# Autodesk Inventor assembly: Y Axis Assembly 1.0_MIR
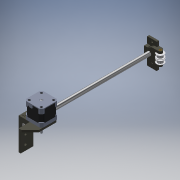
[picture p0: Inventor's stored thumbnail of the model, 180x180]
Saved by Autodesk Inventor 2016 (Build 200138000, 138)
## iProperties
Created: 2017-04-09
Part Number: Y Axis Assembly 1.0_MIR
Document SubType Name: Assembly
Designer: Scott
Author: Scott
## Documents named in this file (11)
- E:\Scott Projects\3D Printing\CoreXY\Y Axis Assembly 1.0_MIR.iam
- E:\Scott Projects\3D Printing\CoreXY\Linear rail - Y_MIR.ipt
- E:\Scott Projects\3D Printing\CoreXY\XY Idler Mount 1.0_MIR.ipt
- E:\Scott Projects\3D Printing\CoreXY\XY Stepper Mount 1.0_MIR.ipt
- E:\Scott Projects\3D Printing\CoreXY\M3 Threaded Insert_MIR3.ipt
- C:\Users\Scott\Documents\Inventor\Content Center Files\R2016\en-US\ANSI B18.3.1M(1)\ANSI B18.3.1M - M3x0.5 x 20(2).ipt
- C:\Users\Scott\Documents\Inventor\Content Center Files\R2016\en-US\ANSI B18.3.1M(1)\ANSI B18.3.1M - M3x0.5 x 30(2).ipt
- E:\Scott Projects\3D Printing\CoreXY\GT2_20t_wheel_pulley_MIR2.ipt
- C:\Users\Scott\Documents\Inventor\Content Center Files\R2016\en-US\ISO 7089\ISO 7089 - 3 - 140 HV(1).ipt
- C:\Users\Scott\Documents\Inventor\Content Center Files\R2016\en-US\AS 1420\AS 1420 - 1973 - M3 x 12.ipt
- E:\Scott Projects\3D Printing\CoreXY\NEMA 17 Stepper Motor Assembly.iam
## Components (19 placed, 10 different names)
1. Linear rail - Y_MIR:1 — Flush:3, Flush:2, Flush:1, Angle:1, Mate:1, Flush:4, Mate:2, Flush:5
2. XY Idler Mount 1.0_MIR:1 — Angle:1, Mate:1, Flush:4, Angle:2, Insert:2, Insert:3, Insert:5, Insert:6, Insert:7, Insert:8
3. XY Stepper Mount 1.0_MIR:1 — Angle:2, Mate:2, Flush:5, Insert:1, Insert:4, Insert:16, Insert:15, Insert:14, Insert:17, Angle:3
4. M3 Threaded Insert_MIR3:1 — Insert:2
5. M3 Threaded Insert_MIR3:2 — Insert:3
6. M3 Threaded Insert_MIR3:3 — Insert:1
7. Broached Socket Head Cap Screw - Metric M3x0.5 x 20:1 — Insert:4
8. Broached Socket Head Cap Screw - Metric M3x0.5 x 20:2 — Insert:5
9. Broached Socket Head Cap Screw - Metric M3x0.5 x 30:1 — Insert:6
10. GT2_20t_wheel_pulley_MIR2:1 — Insert:7, Insert:9
11. GT2_20t_wheel_pulley_MIR2:2 — Insert:8
12. ISO 7089 3 - 140 HV:1 — Insert:9, Insert:10
13. ISO 7089 3 - 140 HV:2 — Insert:12
14. ISO 7089 3 - 140 HV:3 — Insert:12, Insert:11
15. ISO 7089 3 - 140 HV:4 — Insert:11, Insert:10
16. AS 1420 - Metric M3 x 12:1 — Insert:16
17. AS 1420 - Metric M3 x 12:2 — Insert:15
18. AS 1420 - Metric M3 x 12:3 — Insert:14
19. NEMA 17 Stepper Motor Assembly:1 [sub-assembly] — Insert:17, Angle:3
## Relationships (26: Insert 16, Flush 5, Angle 3, Mate 2)
- Flush:3: Linear rail - Y_MIR:1
- Flush:2: Linear rail - Y_MIR:1
- Flush:1: Linear rail - Y_MIR:1
- Angle:1 (180 deg): Linear rail - Y_MIR:1 ↔ XY Idler Mount 1.0_MIR:1
- Mate:1: Linear rail - Y_MIR:1 ↔ XY Idler Mount 1.0_MIR:1
- Flush:4: Linear rail - Y_MIR:1 ↔ XY Idler Mount 1.0_MIR:1
- Angle:2 (0 deg): XY Idler Mount 1.0_MIR:1 ↔ XY Stepper Mount 1.0_MIR:1
- Mate:2: Linear rail - Y_MIR:1 ↔ XY Stepper Mount 1.0_MIR:1
- Flush:5: Linear rail - Y_MIR:1 ↔ XY Stepper Mount 1.0_MIR:1
- Insert:2: XY Idler Mount 1.0_MIR:1 ↔ M3 Threaded Insert_MIR3:1
- Insert:3: XY Idler Mount 1.0_MIR:1 ↔ M3 Threaded Insert_MIR3:2
- Insert:1: XY Stepper Mount 1.0_MIR:1 ↔ M3 Threaded Insert_MIR3:3
- Insert:4: XY Stepper Mount 1.0_MIR:1 ↔ Broached Socket Head Cap Screw - Metric M3x0.5 x 20:1
- Insert:5: XY Idler Mount 1.0_MIR:1 ↔ Broached Socket Head Cap Screw - Metric M3x0.5 x 20:2
- Insert:6: XY Idler Mount 1.0_MIR:1 ↔ Broached Socket Head Cap Screw - Metric M3x0.5 x 30:1
- Insert:7: XY Idler Mount 1.0_MIR:1 ↔ GT2_20t_wheel_pulley_MIR2:1
- Insert:8: XY Idler Mount 1.0_MIR:1 ↔ GT2_20t_wheel_pulley_MIR2:2
- Insert:9: GT2_20t_wheel_pulley_MIR2:1 ↔ ISO 7089 3 - 140 HV:1
- Insert:12: ISO 7089 3 - 140 HV:2 ↔ ISO 7089 3 - 140 HV:3
- Insert:11: ISO 7089 3 - 140 HV:3 ↔ ISO 7089 3 - 140 HV:4
- Insert:10: ISO 7089 3 - 140 HV:1 ↔ ISO 7089 3 - 140 HV:4
- Insert:16: XY Stepper Mount 1.0_MIR:1 ↔ AS 1420 - Metric M3 x 12:1
- Insert:15: XY Stepper Mount 1.0_MIR:1 ↔ AS 1420 - Metric M3 x 12:2
- Insert:14: XY Stepper Mount 1.0_MIR:1 ↔ AS 1420 - Metric M3 x 12:3
- Insert:17: XY Stepper Mount 1.0_MIR:1 ↔ NEMA 17 Stepper Motor Assembly:1
- Angle:3 (0 deg): XY Stepper Mount 1.0_MIR:1 ↔ NEMA 17 Stepper Motor Assembly:1
